# Autodesk Inventor assembly: SYSTEM-FLANGE
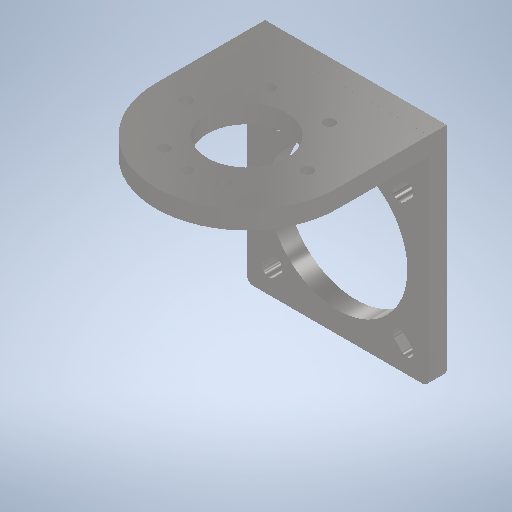
[picture p0: Inventor's stored thumbnail of the model, 512x512]
Saved by Autodesk Inventor 2025.3 (Build 293356030, 356C)
## iProperties
Created: 2025-11-27
Part Number: SYSTEM-FLANGE
Document SubType Name: Assembly
Designer: lstk1ng
Author: lstk1ng
## Documents named in this file (3)
- C:\Users\lstk1ng\Documents\UPC\UPC-10\PROYECTO MECATRONICO 1\DISEÑO MECANICO\SYSTEM-FLANGE.iam
- C:\Users\lstk1ng\Documents\UPC\UPC-10\PROYECTO MECATRONICO 1\DISEÑO MECANICO\SYSTEM-FLANGE-K60.ipt
- C:\Users\lstk1ng\Documents\UPC\UPC-10\PROYECTO MECATRONICO 1\DISEÑO MECANICO\SYSTEM-FLANGE-LOWER.ipt
## Components (2 placed, 2 different names)
1. SYSTEM-FLANGE-K60:1 — Mate:1, Mate:2, Mate:3
2. SYSTEM-FLANGE-LOWER:1 — Mate:1, Mate:2, Mate:3
## Relationships (3: Mate 3)
- Mate:1: SYSTEM-FLANGE-K60:1 ↔ SYSTEM-FLANGE-LOWER:1
- Mate:2: SYSTEM-FLANGE-K60:1 ↔ SYSTEM-FLANGE-LOWER:1
- Mate:3: SYSTEM-FLANGE-K60:1 ↔ SYSTEM-FLANGE-LOWER:1
